# Autodesk Inventor assembly: backpairofwheels
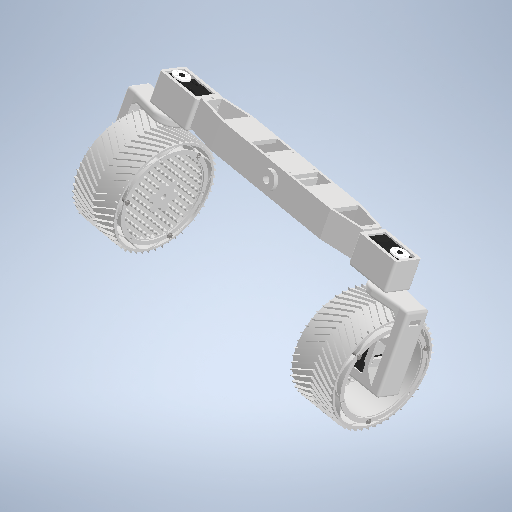
[picture p0: Inventor's stored thumbnail of the model, 512x512]
Saved by Autodesk Inventor 2025.3 (Build 293356000, 356)
## iProperties
Created: 2026-04-12
Part Number: backpairofwheels
Document SubType Name: Assembly
Designer: ksawe
Author: ksawe
## Documents named in this file (4)
- C:\Users\ksawe\OneDrive\Pulpit\Exomy v1\wersja2\backpairofwheels.iam
- C:\Users\ksawe\OneDrive\Pulpit\Exomy v1\wersja2\pret_handler_v2.ipt
- C:\Users\ksawe\OneDrive\Pulpit\Exomy v1\wersja2\wheelbasketback.iam
- C:\Users\ksawe\OneDrive\Pulpit\Exomy v1\wersja2\nakladka.ipt
## Components (4 placed, 3 different names)
1. pret_handler_v2:1 — Mate:1, Mate:2, Mate:3, Mate:4, Mate:5, Mate:6, Mate:7, Mate:8, Mate:9
2. wheelbasketback:1 [sub-assembly] — Mate:1, Mate:3, Mate:4
3. wheelbasketback:2 [sub-assembly] — Mate:2, Mate:5, Mate:6
4. nakladka:1 — Mate:7, Mate:8, Mate:9
## Relationships (9: Mate 9)
- Mate:1: pret_handler_v2:1 ↔ wheelbasketback:1
- Mate:2: pret_handler_v2:1 ↔ wheelbasketback:2
- Mate:3: pret_handler_v2:1 ↔ wheelbasketback:1
- Mate:4: pret_handler_v2:1 ↔ wheelbasketback:1
- Mate:5: pret_handler_v2:1 ↔ wheelbasketback:2
- Mate:6: pret_handler_v2:1 ↔ wheelbasketback:2
- Mate:7: pret_handler_v2:1 ↔ nakladka:1
- Mate:8: pret_handler_v2:1 ↔ nakladka:1
- Mate:9: pret_handler_v2:1 ↔ nakladka:1
